# Autodesk Inventor assembly: Plank Assembly
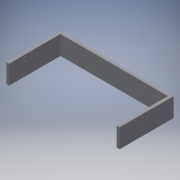
[picture p0: Inventor's stored thumbnail of the model, 180x180]
Saved by Autodesk Inventor 2018 (Build 220112000, 112)
## iProperties
Created: 2020-01-25
Part Number: Plank Assembly
Document SubType Name: Assembly
Designer: S-2512711
Author: S-2512711
## Documents named in this file (3)
- \\studenthome\students\S-2512711\GitHub\2020CAD\Bumpers\Part Files\Plank Assembly.iam
- \\studenthome\students\S-2512711\GitHub\2020CAD\Bumpers\Part Files\Long Plank.ipt
- \\studenthome\students\S-2512711\GitHub\2020CAD\Bumpers\Part Files\Short Plank.ipt
## Components (3 placed, 2 different names)
1. Long Plank:1 — Mate:1, Flush:1, Flush:2, Flush:3, Flush:4, Mate:2
2. Short Plank:1 — Mate:1, Flush:1, Flush:2
3. Short Plank:2 — Flush:3, Flush:4, Mate:2
## Relationships (6: Flush 4, Mate 2)
- Mate:1: Long Plank:1 ↔ Short Plank:1
- Flush:1: Long Plank:1 ↔ Short Plank:1
- Flush:2: Long Plank:1 ↔ Short Plank:1
- Flush:3: Long Plank:1 ↔ Short Plank:2
- Flush:4: Long Plank:1 ↔ Short Plank:2
- Mate:2: Long Plank:1 ↔ Short Plank:2
